# Autodesk Inventor assembly: NeoClock
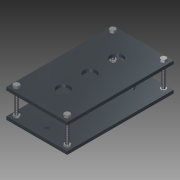
[picture p0: Inventor's stored thumbnail of the model, 180x180]
Saved by Autodesk Inventor 2015 (Build 190159000, 159)
## iProperties
Created: 2015-09-07
Part Number: NeoClock
Document SubType Name: Assembly
Designer: Silas
Author: Silas
## Documents named in this file (6)
- D:\Dropbox\silas_og_tobias\3D Printer\inventor\NeoClock\NeoClock.iam
- D:\Dropbox\silas_og_tobias\3D Printer\inventor\NeoClock\Back cover.ipt
- D:\Dropbox\silas_og_tobias\3D Printer\inventor\NeoClock\Front cover.ipt
- D:\Documents\Inventor\Content Center Files\R2015\en-US\ANSI B 18.6.7 M IFI 513(5)\ANSI B 18.6.7 M _ IFI 513 - M3 x 0,5 x 30(3).ipt
- D:\Documents\Inventor\Content Center Files\R2015\en-US\JIS B 1181  A B\JIS B 1181 - A_B M2,5.ipt
- D:\Documents\Inventor\Content Center Files\R2015\en-US\JIS B 1181  A B\JIS B 1181 - A_B M3.ipt
## Components (18 placed, 5 different names)
1. Trimmed Hex Head Machine Screw - Metric M3 x 0,5 x 30:1 — Insert:2, Insert:11
2. Trimmed Hex Head Machine Screw - Metric M3 x 0,5 x 30:2 — Insert:1, Insert:12
3. Trimmed Hex Head Machine Screw - Metric M3 x 0,5 x 30:3 — Insert:4, Insert:9
4. Trimmed Hex Head Machine Screw - Metric M3 x 0,5 x 30:4 — Insert:3, Insert:10
5. Back cover:1 — Insert:13, Insert:14, Insert:17, Insert:18, Insert:19
6. Front cover:1 — Insert:1, Insert:2, Insert:3, Insert:4, Insert:5, Insert:6, Insert:7, Insert:8
7. JIS B 1181 A/B - Metric A/B M2,5:1 — Insert:5
8. JIS B 1181 A/B - Metric A/B M2,5:2 — Insert:6
9. JIS B 1181 A/B - Metric A/B M2,5:3 — Insert:7
10. JIS B 1181 A/B - Metric A/B M2,5:4 — Insert:8
11. JIS B 1181 A/B - Metric A/B M3:1 — Insert:11
12. JIS B 1181 A/B - Metric A/B M3:2 — Insert:12
13. JIS B 1181 A/B - Metric A/B M3:3 — Insert:10, Insert:13
14. JIS B 1181 A/B - Metric A/B M3:4 — Insert:9
15. JIS B 1181 A/B - Metric A/B M2,5:5 — Insert:14
16. JIS B 1181 A/B - Metric A/B M2,5:8 — Insert:17
17. JIS B 1181 A/B - Metric A/B M2,5:9 — Insert:18
18. JIS B 1181 A/B - Metric A/B M2,5:10 — Insert:19
## Relationships (17: Insert 17)
- Insert:1: Trimmed Hex Head Machine Screw - Metric M3 x 0,5 x 30:2 ↔ Front cover:1
- Insert:2: Trimmed Hex Head Machine Screw - Metric M3 x 0,5 x 30:1 ↔ Front cover:1
- Insert:3: Trimmed Hex Head Machine Screw - Metric M3 x 0,5 x 30:4 ↔ Front cover:1
- Insert:4: Trimmed Hex Head Machine Screw - Metric M3 x 0,5 x 30:3 ↔ Front cover:1
- Insert:5: Front cover:1 ↔ JIS B 1181 A/B - Metric A/B M2,5:1
- Insert:6: Front cover:1 ↔ JIS B 1181 A/B - Metric A/B M2,5:2
- Insert:7: Front cover:1 ↔ JIS B 1181 A/B - Metric A/B M2,5:3
- Insert:8: Front cover:1 ↔ JIS B 1181 A/B - Metric A/B M2,5:4
- Insert:9: Trimmed Hex Head Machine Screw - Metric M3 x 0,5 x 30:3 ↔ JIS B 1181 A/B - Metric A/B M3:4
- Insert:10: Trimmed Hex Head Machine Screw - Metric M3 x 0,5 x 30:4 ↔ JIS B 1181 A/B - Metric A/B M3:3
- Insert:11: Trimmed Hex Head Machine Screw - Metric M3 x 0,5 x 30:1 ↔ JIS B 1181 A/B - Metric A/B M3:1
- Insert:12: Trimmed Hex Head Machine Screw - Metric M3 x 0,5 x 30:2 ↔ JIS B 1181 A/B - Metric A/B M3:2
- Insert:13: Back cover:1 ↔ JIS B 1181 A/B - Metric A/B M3:3
- Insert:14: Back cover:1 ↔ JIS B 1181 A/B - Metric A/B M2,5:5
- Insert:17: Back cover:1 ↔ JIS B 1181 A/B - Metric A/B M2,5:8
- Insert:18: Back cover:1 ↔ JIS B 1181 A/B - Metric A/B M2,5:9
- Insert:19: Back cover:1 ↔ JIS B 1181 A/B - Metric A/B M2,5:10
